# Autodesk Inventor assembly: Hexagonal Deco Lamp Assembly 150
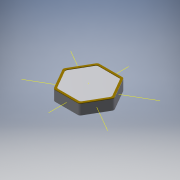
[picture p0: Inventor's stored thumbnail of the model, 180x180]
Saved by Autodesk Inventor 2019 (Build 230136000, 136)
## iProperties
Created: 2021-07-14
Part Number: Hexagonal Deco Lamp Assembly 150
Document SubType Name: Assembly
Designer: Lix
Author: Lix
## Documents named in this file (4)
- G:\Project\Hybrids\HexaWall\Inventor\Hexagonal Deco Lamp Assembly 175.iam
- G:\Project\Hybrids\HexaWall\Inventor\Frosted Top v1 - 175.ipt
- G:\Project\Hybrids\HexaWall\Inventor\Cover v1 - 175 - 8mm rim.ipt
- G:\Project\Hybrids\HexaWall\Inventor\Base v6 - 175.ipt
## Components (3 placed, 3 different names)
1. Base v6 - 175:1 — Flush:2, Flush:3, Mate:5, Flush:4
2. Cover v1 - 175 - 8mm rim:1 — Flush:2, Flush:3, Mate:5, Flush:4, Mate:6, Mate:7, Mate:8
3. Frosted Top v1 - 175:1 — Mate:6, Mate:7, Mate:8
## Relationships (7: Mate 4, Flush 3)
- Flush:2: Base v6 - 175:1 ↔ Cover v1 - 175 - 8mm rim:1
- Flush:3: Base v6 - 175:1 ↔ Cover v1 - 175 - 8mm rim:1
- Mate:5: Base v6 - 175:1 ↔ Cover v1 - 175 - 8mm rim:1
- Flush:4: Base v6 - 175:1 ↔ Cover v1 - 175 - 8mm rim:1
- Mate:6: Cover v1 - 175 - 8mm rim:1 ↔ Frosted Top v1 - 175:1
- Mate:7: Cover v1 - 175 - 8mm rim:1 ↔ Frosted Top v1 - 175:1
- Mate:8: Cover v1 - 175 - 8mm rim:1 ↔ Frosted Top v1 - 175:1
